# Autodesk Inventor assembly: Dumber_2022
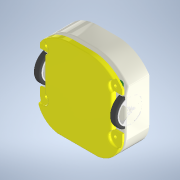
[picture p0: Inventor's stored thumbnail of the model, 180x180]
Saved by Autodesk Inventor 2021 (Build 250183000, 183)
## iProperties
Created: 2022-05-24
Part Number: Dumber_2022
Document SubType Name: Assembly
Designer: dimercur
Author: dimercur
## Documents named in this file (5)
- C:\Users\dimercur\Documents\Projets Git\dumber\hardware\meca\Dumber_2022\Dumber_2022.iam
- C:\Users\dimercur\Documents\Projets Git\dumber\hardware\meca\Dumber_2022\Pieces\pcb.ipt
- C:\Users\dimercur\Documents\Projets Git\dumber\hardware\meca\Dumber_2022\Pieces\moteur.iam
- C:\Users\dimercur\Documents\Projets Git\dumber\hardware\meca\Dumber_2022\Pieces\roue.iam
- C:\Users\dimercur\Documents\Projets Git\dumber\hardware\meca\Dumber_2022\Pieces\coque_inf.ipt
## Components (6 placed, 4 different names)
1. pcb:1 — Placage:1, Placage:2, Placage:3, Placage:4, Placage:5, Placage:6, Placage:11, Placage:12, Placage:13
2. moteur:1 [sub-assembly] — Placage:1, Placage:3, Placage:4, Placage:7, Placage:9, Affleurement:2
3. roue:1 [sub-assembly] — Placage:8, Placage:10, Affleurement:1
4. moteur:2 [sub-assembly] — Placage:2, Placage:5, Placage:6, Placage:8, Placage:10, Affleurement:1
5. roue:2 [sub-assembly] — Placage:7, Placage:9, Affleurement:2
6. coque_inf:1 — Placage:11, Placage:12, Placage:13
## Relationships (15: Mate 13, Flush 2)
- Placage:1 [Mate]: pcb:1 ↔ moteur:1
- Placage:2 [Mate]: pcb:1 ↔ moteur:2
- Placage:3 [Mate]: pcb:1 ↔ moteur:1
- Placage:4 [Mate]: pcb:1 ↔ moteur:1
- Placage:5 [Mate]: pcb:1 ↔ moteur:2
- Placage:6 [Mate]: pcb:1 ↔ moteur:2
- Placage:7 [Mate]: moteur:1 ↔ roue:2
- Placage:8 [Mate]: roue:1 ↔ moteur:2
- Placage:9 [Mate]: moteur:1 ↔ roue:2
- Placage:10 [Mate]: roue:1 ↔ moteur:2
- Affleurement:1 [Flush]: roue:1 ↔ moteur:2
- Affleurement:2 [Flush]: moteur:1 ↔ roue:2
- Placage:11 [Mate]: pcb:1 ↔ coque_inf:1
- Placage:12 [Mate]: pcb:1 ↔ coque_inf:1
- Placage:13 [Mate]: pcb:1 ↔ coque_inf:1
